# Autodesk Inventor assembly: Gen 2.0 Robot
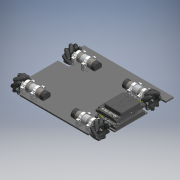
[picture p0: Inventor's stored thumbnail of the model, 180x180]
Saved by Autodesk Inventor 2019 (Build 230136000, 136)
## iProperties
Part Number: Gen 2.0 Robot
Document SubType Name: Assembly
Designer: Delta
Author: Delta
## Documents named in this file (8)
- C:\Robotics\2019-20_CAD\Drive Train\Gen 2.0 Robot.iam
- C:\Robotics\2019-20_CAD\Drive Train\Gen 2.0 rev mecanums base plate.ipt
- C:\Robotics\COTSParts\Motors\am-3102NeveRest20 (1).ipt
- C:\Robotics\COTSParts\Tetrix\tetrix-motor-mounts-1.snapshot.1\Tetrex 2pc motor mount.ipt
- C:\Robotics\COTSParts\Rev\REV-31-1153RevHub.ipt
- C:\Robotics\COTSParts\Rev\REV-41-1656MecanumWheel.iam
- C:\Robotics\COTSParts\Rev\REV-41-1657MecanumWheelRight.iam
- C:\Robotics\COTSParts\Tetrix\Tetrix hub - motor.ipt
## Components (23 placed, 7 different names)
1. Gen 2.0 rev mecanums base plate:1 — Mate:1, Mate:2, Flush:7, Mate:4, Flush:8, Mate:5, Mate:7, Mate:8, Mate:10, Flush:17, Flush:18, Mate:11, Mate:13, Mate:14, Angle:1, Angle:2, Angle:3, Angle:4, Flush:21, Flush:22, Flush:23, Flush:24, Mate:44, Mate:45, Mate:46, Mate:48
2. am-3102NeveRest20 (1):1 — Mate:12, Flush:19, Flush:20, Mate:36, Mate:37, Angle:2
3. am-3102NeveRest20 (1):2 — Mate:9, Flush:14, Flush:15, Mate:31, Mate:32, Angle:3, Mate:43
4. am-3102NeveRest20 (1):3 — Mate:3, Flush:4, Flush:5, Mate:21, Mate:22, Angle:4, Mate:42
5. am-3102NeveRest20 (1):4 — Mate:6, Flush:9, Flush:10, Mate:26, Mate:27, Angle:1
6. Tetrex 2pc motor mount:1 — Mate:2, Flush:5, Mate:42
7. Tetrex 2pc motor mount:2 — Mate:1, Mate:3, Flush:4, Flush:21, Mate:44
8. Tetrex 2pc motor mount:3 — Mate:8, Flush:15, Mate:43
9. Tetrex 2pc motor mount:4 — Mate:7, Mate:9, Flush:14, Flush:22, Mate:45
10. Tetrex 2pc motor mount:5 — Mate:10, Flush:17, Mate:12, Flush:19, Flush:23
11. Tetrex 2pc motor mount:6 — Flush:18, Mate:11, Flush:20
12. Tetrex 2pc motor mount:7 — Flush:8, Mate:5, Flush:10
13. Tetrex 2pc motor mount:8 — Flush:7, Mate:4, Mate:6, Flush:9, Flush:24
14. REV-31-1153RevHub:1 — Mate:13, Mate:14, Mate:46, Mate:47, Mate:49
15. REV-31-1153RevHub:2 — Mate:47, Mate:48, Mate:49
16. REV-41-1656MecanumWheel:1 [sub-assembly] — Mate:28, Mate:29, Mate:30
17. REV-41-1656MecanumWheel:2 [sub-assembly] — Mate:23, Mate:24, Mate:25
18. REV-41-1657MecanumWheelRight:1 [sub-assembly] — Mate:33, Mate:34, Mate:35
19. REV-41-1657MecanumWheelRight:2 [sub-assembly] — Mate:18, Mate:19, Mate:20
20. Tetrix hub - motor:1 — Mate:18, Mate:19, Mate:20, Mate:21, Mate:22
21. Tetrix hub - motor:2 — Mate:23, Mate:24, Mate:25, Mate:26, Mate:27
22. Tetrix hub - motor:3 — Mate:33, Mate:34, Mate:35, Mate:36, Mate:37
23. Tetrix hub - motor:4 — Mate:28, Mate:29, Mate:30, Mate:31, Mate:32
## Relationships (62: Mate 42, Flush 16, Angle 4)
- Mate:1: Gen 2.0 rev mecanums base plate:1 ↔ Tetrex 2pc motor mount:2
- Mate:2: Gen 2.0 rev mecanums base plate:1 ↔ Tetrex 2pc motor mount:1
- Mate:3: am-3102NeveRest20 (1):3 ↔ Tetrex 2pc motor mount:2
- Flush:4: am-3102NeveRest20 (1):3 ↔ Tetrex 2pc motor mount:2
- Flush:5: am-3102NeveRest20 (1):3 ↔ Tetrex 2pc motor mount:1
- Flush:7: Gen 2.0 rev mecanums base plate:1 ↔ Tetrex 2pc motor mount:8
- Mate:4: Gen 2.0 rev mecanums base plate:1 ↔ Tetrex 2pc motor mount:8
- Flush:8: Gen 2.0 rev mecanums base plate:1 ↔ Tetrex 2pc motor mount:7
- Mate:5: Gen 2.0 rev mecanums base plate:1 ↔ Tetrex 2pc motor mount:7
- Mate:6: am-3102NeveRest20 (1):4 ↔ Tetrex 2pc motor mount:8
- Flush:9: am-3102NeveRest20 (1):4 ↔ Tetrex 2pc motor mount:8
- Flush:10: am-3102NeveRest20 (1):4 ↔ Tetrex 2pc motor mount:7
- Mate:7: Gen 2.0 rev mecanums base plate:1 ↔ Tetrex 2pc motor mount:4
- Mate:8: Gen 2.0 rev mecanums base plate:1 ↔ Tetrex 2pc motor mount:3
- Mate:9: am-3102NeveRest20 (1):2 ↔ Tetrex 2pc motor mount:4
- Flush:14: am-3102NeveRest20 (1):2 ↔ Tetrex 2pc motor mount:4
- Flush:15: am-3102NeveRest20 (1):2 ↔ Tetrex 2pc motor mount:3
- Mate:10: Gen 2.0 rev mecanums base plate:1 ↔ Tetrex 2pc motor mount:5
- Flush:17: Gen 2.0 rev mecanums base plate:1 ↔ Tetrex 2pc motor mount:5
- Flush:18: Gen 2.0 rev mecanums base plate:1 ↔ Tetrex 2pc motor mount:6
- Mate:11: Gen 2.0 rev mecanums base plate:1 ↔ Tetrex 2pc motor mount:6
- Mate:12: am-3102NeveRest20 (1):1 ↔ Tetrex 2pc motor mount:5
- Flush:19: am-3102NeveRest20 (1):1 ↔ Tetrex 2pc motor mount:5
- Flush:20: am-3102NeveRest20 (1):1 ↔ Tetrex 2pc motor mount:6
- Mate:13: Gen 2.0 rev mecanums base plate:1 ↔ REV-31-1153RevHub:1
- Mate:14: Gen 2.0 rev mecanums base plate:1 ↔ REV-31-1153RevHub:1
- Mate:18: REV-41-1657MecanumWheelRight:2 ↔ Tetrix hub - motor:1
- Mate:19: REV-41-1657MecanumWheelRight:2 ↔ Tetrix hub - motor:1
- Mate:20: REV-41-1657MecanumWheelRight:2 ↔ Tetrix hub - motor:1
- Mate:21: am-3102NeveRest20 (1):3 ↔ Tetrix hub - motor:1
- Mate:22 (6.35 mm): am-3102NeveRest20 (1):3 ↔ Tetrix hub - motor:1
- Mate:23: REV-41-1656MecanumWheel:2 ↔ Tetrix hub - motor:2
- Mate:24: REV-41-1656MecanumWheel:2 ↔ Tetrix hub - motor:2
- Mate:25: REV-41-1656MecanumWheel:2 ↔ Tetrix hub - motor:2
- Mate:26: am-3102NeveRest20 (1):4 ↔ Tetrix hub - motor:2
- Mate:27 (6.35 mm): am-3102NeveRest20 (1):4 ↔ Tetrix hub - motor:2
- Mate:28: REV-41-1656MecanumWheel:1 ↔ Tetrix hub - motor:4
- Mate:29: REV-41-1656MecanumWheel:1 ↔ Tetrix hub - motor:4
- Mate:30: REV-41-1656MecanumWheel:1 ↔ Tetrix hub - motor:4
- Mate:31 (6.35 mm): am-3102NeveRest20 (1):2 ↔ Tetrix hub - motor:4
- Mate:32: am-3102NeveRest20 (1):2 ↔ Tetrix hub - motor:4
- Mate:33: REV-41-1657MecanumWheelRight:1 ↔ Tetrix hub - motor:3
- Mate:34: REV-41-1657MecanumWheelRight:1 ↔ Tetrix hub - motor:3
- Mate:35: REV-41-1657MecanumWheelRight:1 ↔ Tetrix hub - motor:3
- Mate:36 (6.35 mm): am-3102NeveRest20 (1):1 ↔ Tetrix hub - motor:3
- Mate:37: am-3102NeveRest20 (1):1 ↔ Tetrix hub - motor:3
- Angle:1 (180 deg): Gen 2.0 rev mecanums base plate:1 ↔ am-3102NeveRest20 (1):4
- Angle:2 (180 deg): Gen 2.0 rev mecanums base plate:1 ↔ am-3102NeveRest20 (1):1
- Angle:3 (180 deg): Gen 2.0 rev mecanums base plate:1 ↔ am-3102NeveRest20 (1):2
- Angle:4 (180 deg): Gen 2.0 rev mecanums base plate:1 ↔ am-3102NeveRest20 (1):3
- Flush:21: Gen 2.0 rev mecanums base plate:1 ↔ Tetrex 2pc motor mount:2
- Mate:42: am-3102NeveRest20 (1):3 ↔ Tetrex 2pc motor mount:1
- Flush:22: Gen 2.0 rev mecanums base plate:1 ↔ Tetrex 2pc motor mount:4
- Mate:43: am-3102NeveRest20 (1):2 ↔ Tetrex 2pc motor mount:3
- Flush:23: Gen 2.0 rev mecanums base plate:1 ↔ Tetrex 2pc motor mount:5
- Flush:24: Gen 2.0 rev mecanums base plate:1 ↔ Tetrex 2pc motor mount:8
- Mate:44 (12.7 mm): Gen 2.0 rev mecanums base plate:1 ↔ Tetrex 2pc motor mount:2
- Mate:45 (12.7 mm): Gen 2.0 rev mecanums base plate:1 ↔ Tetrex 2pc motor mount:4
- Mate:46 (-6.35 mm): Gen 2.0 rev mecanums base plate:1 ↔ REV-31-1153RevHub:1
- Mate:47: REV-31-1153RevHub:1 ↔ REV-31-1153RevHub:2
- Mate:48: Gen 2.0 rev mecanums base plate:1 ↔ REV-31-1153RevHub:2
- Mate:49: REV-31-1153RevHub:1 ↔ REV-31-1153RevHub:2
